# Autodesk Inventor assembly: IndexBeltSys
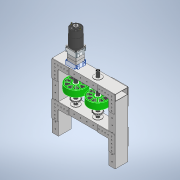
[picture p0: Inventor's stored thumbnail of the model, 180x180]
Saved by Autodesk Inventor 2022 (Build 260153000, 153)
## iProperties
Created: 2022-01-13
Part Number: IndexBeltSys
Document SubType Name: Assembly
Designer: tagaz
Author: tagaz
## Documents named in this file (12)
- C:\Users\tagaz\OneDrive\Documents\T3-Cad\CAD\2022 Parts\IndexBeltSys.iam
- IndexSys.iam
- C:\Users\tagaz\OneDrive\Documents\T3-Cad\CAD\2022 Parts\Generic\VersaFrame_IndexSupp.ipt
- C:\Users\tagaz\OneDrive\Documents\T3-Cad\CAD\2022 Parts\Generic\VersaFrame_VelcRail.ipt
- C:\Users\tagaz\OneDrive\Documents\T3-Cad\CAD\Generic and Stock\VersaGusset 90o.ipt
- C:\Users\tagaz\OneDrive\Documents\T3-Cad\CAD\Bearing  for THUNDER.ipt
- C:\Users\tagaz\OneDrive\Documents\T3-Cad\CAD\Generic and Stock\VersaPlanetary Parts\VersaPlanetary Two Stage 775.iam
- C:\Users\tagaz\OneDrive\Documents\T3-Cad\CAD\2022 Parts\Generic\VersaFrame_VelcRail2.ipt
- C:\Users\tagaz\OneDrive\Documents\T3-Cad\CAD\2022 Parts\Generic\indexThundershaft.ipt
- C:\Users\tagaz\OneDrive\Documents\T3-Cad\CAD\2022 Parts\Generic\indexThundershaft2.ipt
- C:\Users\tagaz\OneDrive\Documents\T3-Cad\CAD\2022 Parts\16T Alum Hub Sprock 25 Chain.ipt
- C:\Users\tagaz\OneDrive\Documents\T3-Cad\CAD\2022 Parts\Generic\3in Compliance wheel.ipt
## Components (26 placed, 10 different names)
1. VersaFrame_IndexSupp:1 — Flush:5, Flush:6, Mate:3, Flush:8, Flush:9, Flush:24, Mate:31
2. VersaFrame_IndexSupp:2 — Mate:2, Flush:3, Flush:4, Mate:6, Flush:12, Mate:7
3. VersaFrame_VelcRail:1 — Mate:2, Flush:3, Flush:4, Flush:5, Flush:6, Mate:3, Flush:7, Mate:4, Mate:5, Flush:10, Flush:11, Flush:13, Flush:14, Mate:8, Insert:1, Insert:2, Insert:3, Mate:30, Flush:27, Mate:40, Mate:54, Mate:55
4. Bearing  for THUNDER:1 — Insert:3, Mate:41
5. Bearing  for THUNDER:2 — Insert:2
6. Bearing  for THUNDER:5 — Mate:8, Insert:1
7. Bearing  for THUNDER:7 — Insert:6, Mate:38, Mate:39
8. Bearing  for THUNDER:8 — Insert:7
9. VersaPlanetary Two Stage 775:1 [sub-assembly] — Flush:27, Mate:40, Mate:41
10. VersaFrame_VelcRail2:1 — Flush:24, Mate:30, Mate:31, Insert:6, Insert:7, Insert:8, Insert:9
11. indexThundershaft:2 — Flush:26, Mate:38, Mate:39, Mate:48, Mate:49, Mate:52, Mate:53
12. Bearing  for THUNDER:9 — Insert:9, Flush:26
13. Bearing  for THUNDER:10 — Insert:8, Flush:28, Mate:42, Mate:43
14. indexThundershaft2:1 — Flush:28, Mate:42, Mate:43, Mate:45, Mate:46, Mate:50, Mate:51
15. 16T Alum Hub Sprock 25 Chain:4 — Mate:45, Mate:46
16. 16T Alum Hub Sprock 25 Chain:5 — Mate:48, Mate:49
17. 3in Compliance wheel:1 — Mate:50, Mate:51, Mate:55
18. 3in Compliance wheel:2 — Mate:52, Mate:53, Mate:54
19. VersaGusset 90o:4 — Mate:6, Flush:11, Flush:12
20. VersaGusset 90o:3 — Mate:7, Flush:13, Flush:14
21. VersaGusset 90o:1 — Mate:5, Flush:9, Flush:10
22. VersaGusset 90o:2 — Flush:7, Mate:4, Flush:8
23. VersaGusset 90o:5
24. VersaGusset 90o:6
25. VersaGusset 90o:7
26. VersaGusset 90o:8
## Component patterns: (2 elements, first: VersaGusset 90o:4 + VersaGusset 90o:3 + VersaGusset 90o:1 + VersaGusset 90o:2)
## Relationships (48: Mate 25, Flush 16, Insert 7)
- Mate:2: VersaFrame_IndexSupp:2 ↔ VersaFrame_VelcRail:1
- Flush:3: VersaFrame_IndexSupp:2 ↔ VersaFrame_VelcRail:1
- Flush:4: VersaFrame_IndexSupp:2 ↔ VersaFrame_VelcRail:1
- Flush:5: VersaFrame_IndexSupp:1 ↔ VersaFrame_VelcRail:1
- Flush:6: VersaFrame_IndexSupp:1 ↔ VersaFrame_VelcRail:1
- Mate:3: VersaFrame_IndexSupp:1 ↔ VersaFrame_VelcRail:1
- Flush:7: VersaFrame_VelcRail:1 ↔ VersaGusset 90o:2
- Mate:4: VersaFrame_VelcRail:1 ↔ VersaGusset 90o:2
- Flush:8: VersaFrame_IndexSupp:1 ↔ VersaGusset 90o:2
- Mate:5: VersaFrame_VelcRail:1 ↔ VersaGusset 90o:1
- Flush:9: VersaFrame_IndexSupp:1 ↔ VersaGusset 90o:1
- Flush:10: VersaFrame_VelcRail:1 ↔ VersaGusset 90o:1
- Mate:6: VersaFrame_IndexSupp:2 ↔ VersaGusset 90o:4
- Flush:11: VersaFrame_VelcRail:1 ↔ VersaGusset 90o:4
- Flush:12: VersaFrame_IndexSupp:2 ↔ VersaGusset 90o:4
- Mate:7: VersaFrame_IndexSupp:2 ↔ VersaGusset 90o:3
- Flush:13: VersaFrame_VelcRail:1 ↔ VersaGusset 90o:3
- Flush:14: VersaFrame_VelcRail:1 ↔ VersaGusset 90o:3
- Mate:8: VersaFrame_VelcRail:1 ↔ Bearing  for THUNDER:5
- Insert:1: VersaFrame_VelcRail:1 ↔ Bearing  for THUNDER:5
- Insert:2: VersaFrame_VelcRail:1 ↔ Bearing  for THUNDER:2
- Insert:3: VersaFrame_VelcRail:1 ↔ Bearing  for THUNDER:1
- Flush:24: VersaFrame_IndexSupp:1 ↔ VersaFrame_VelcRail2:1
- Mate:30 (114.3 mm): VersaFrame_VelcRail:1 ↔ VersaFrame_VelcRail2:1
- Mate:31: VersaFrame_IndexSupp:1 ↔ VersaFrame_VelcRail2:1
- Insert:6: Bearing  for THUNDER:7 ↔ VersaFrame_VelcRail2:1
- Insert:7: Bearing  for THUNDER:8 ↔ VersaFrame_VelcRail2:1
- Flush:26: indexThundershaft:2 ↔ Bearing  for THUNDER:9
- Mate:38: Bearing  for THUNDER:7 ↔ indexThundershaft:2
- Mate:39: Bearing  for THUNDER:7 ↔ indexThundershaft:2
- Flush:27 (4.3942 mm): VersaFrame_VelcRail:1 ↔ VersaPlanetary Two Stage 775:1
- Mate:40: VersaFrame_VelcRail:1 ↔ VersaPlanetary Two Stage 775:1
- Mate:41: Bearing  for THUNDER:1 ↔ VersaPlanetary Two Stage 775:1
- Insert:8: VersaFrame_VelcRail2:1 ↔ Bearing  for THUNDER:10
- Insert:9: VersaFrame_VelcRail2:1 ↔ Bearing  for THUNDER:9
- Flush:28: Bearing  for THUNDER:10 ↔ indexThundershaft2:1
- Mate:42: Bearing  for THUNDER:10 ↔ indexThundershaft2:1
- Mate:43: Bearing  for THUNDER:10 ↔ indexThundershaft2:1
- Mate:45: indexThundershaft2:1 ↔ 16T Alum Hub Sprock 25 Chain:4
- Mate:46: indexThundershaft2:1 ↔ 16T Alum Hub Sprock 25 Chain:4
- Mate:48: indexThundershaft:2 ↔ 16T Alum Hub Sprock 25 Chain:5
- Mate:49: indexThundershaft:2 ↔ 16T Alum Hub Sprock 25 Chain:5
- Mate:50: indexThundershaft2:1 ↔ 3in Compliance wheel:1
- Mate:51: indexThundershaft2:1 ↔ 3in Compliance wheel:1
- Mate:52: indexThundershaft:2 ↔ 3in Compliance wheel:2
- Mate:53: indexThundershaft:2 ↔ 3in Compliance wheel:2
- Mate:54 (38.1 mm): VersaFrame_VelcRail:1 ↔ 3in Compliance wheel:2
- Mate:55 (38.1 mm): VersaFrame_VelcRail:1 ↔ 3in Compliance wheel:1
